# Autodesk Inventor assembly: Full Wheel (H)
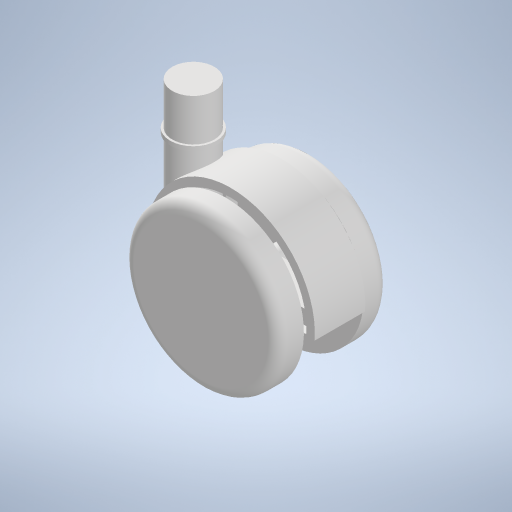
[picture p0: Inventor's stored thumbnail of the model, 512x512]
Saved by Autodesk Inventor 2023 (Build 270158030, 158C)
## iProperties
Created: 2023-03-03
Part Number: Full Wheel (H)
Document SubType Name: Assembly
Designer: mpino
Author: mpino
## Documents named in this file (3)
- C:\Users\mpino\Desktop\Cad\Full Wheel (H).iam
- C:\Users\mpino\Desktop\Cad\Wheel sheild (H).ipt
- C:\Users\mpino\Desktop\Cad\Chairs Wheel (H).ipt
## Components (3 placed, 2 different names)
1. Wheel sheild (H):1 — Mate:1, Mate:2, Mate:3, Mate:4
2. Chairs Wheel (H):1 — Mate:2, Mate:3
3. Chairs Wheel (H):2 — Mate:1, Mate:4
## Relationships (4: Mate 4)
- Mate:1: Wheel sheild (H):1 ↔ Chairs Wheel (H):2
- Mate:2: Wheel sheild (H):1 ↔ Chairs Wheel (H):1
- Mate:3: Wheel sheild (H):1 ↔ Chairs Wheel (H):1
- Mate:4: Wheel sheild (H):1 ↔ Chairs Wheel (H):2
